# Autodesk Inventor assembly: Gehäuse_1
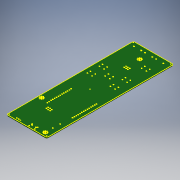
[picture p0: Inventor's stored thumbnail of the model, 180x180]
Saved by Autodesk Inventor 2019 (Build 230136000, 136)
## iProperties
Created: 2018-07-30
Part Number: Gehäuse_1
Material: Generisch
Document SubType Name: Assembly
Designer: marc
Author: marc
## Documents named in this file (3)
- C:\Users\marc\Google Drive\Projekte\fantimote\seniors Remote\seniorsRemote\case\Gehäuse_1.iam
- C:\Users\marc\Google Drive\Projekte\fantimote\seniors Remote\seniorsRemote\pcb\fantimote.kicad_pcb.iam
- C:\Users\marc\Google Drive\Projekte\fantimote\seniors Remote\seniorsRemote\case\Oberschale.ipt
## Components (2 placed, 2 different names)
1. fantimote.kicad_pcb:1 [sub-assembly] — Fluchtend:1
2. Oberschale:1 — Fluchtend:1
## Relationships (1: Flush 1)
- Fluchtend:1 [Flush]: fantimote.kicad_pcb:1 ↔ Oberschale:1
